# Autodesk Inventor assembly: nc_nhk2
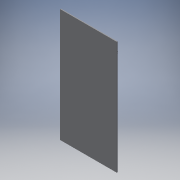
[picture p0: Inventor's stored thumbnail of the model, 180x180]
Saved by Autodesk Inventor 2019 (Build 230136000, 136)
## iProperties
Created: 2022-02-26
Part Number: nc_nhk2
Material: 一般
Document SubType Name: Assembly
Designer: yuta
Author: yuta
## Documents named in this file (3)
- C:\Users\yuta\Documents\NHK\nc_nhk2.iam
- C:\Users\yuta\Documents\NHK\NC.1.ipt
- C:\Users\yuta\Documents\NHK\nhk26.ipt
## Components (4 placed, 2 different names)
1. NC.1:1 — メイト:1, フラッシュ:1, フラッシュ:2, メイト:2, フラッシュ:3, メイト:4, フラッシュ:4, フラッシュ:5
2. nhk26:1 — メイト:2, メイト:3, フラッシュ:3
3. nhk26:2 — メイト:4, フラッシュ:4, フラッシュ:5
4. nhk26:3 — メイト:1, フラッシュ:1, フラッシュ:2, メイト:3
## Relationships (9: Flush 5, Mate 4)
- メイト:1 [Mate]: NC.1:1 ↔ nhk26:3
- フラッシュ:1 [Flush] (45 mm): NC.1:1 ↔ nhk26:3
- フラッシュ:2 [Flush] (50 mm): NC.1:1 ↔ nhk26:3
- メイト:2 [Mate]: NC.1:1 ↔ nhk26:1
- メイト:3 [Mate] (-25 mm): nhk26:1 ↔ nhk26:3
- フラッシュ:3 [Flush] (45 mm): NC.1:1 ↔ nhk26:1
- メイト:4 [Mate]: NC.1:1 ↔ nhk26:2
- フラッシュ:4 [Flush] (45 mm): NC.1:1 ↔ nhk26:2
- フラッシュ:5 [Flush] (30 mm): NC.1:1 ↔ nhk26:2
